# Autodesk Inventor assembly: BG301_trajan20_21
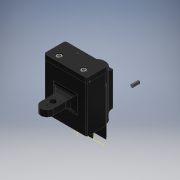
[picture p0: Inventor's stored thumbnail of the model, 180x180]
Saved by Autodesk Inventor 2022.2 (Build 262287000, 287)
## iProperties
Company: HTBLA Kaindorf
RuleStatus: InUse
Created: 2022-08-19
Part Number: BG301_trajan20_21
Project: Zeichenmaschine_v2
Material: Generisch
Description: Stifthalter
Document SubType Name: Assembly
Designer: trajan20
AfterDocNew0: iProperties-Editor_aufrufen
Author: jan
Keywords: 2021
## Documents named in this file (7)
- C:\Users\jan\Documents\DrawMachine\DrawMachineConstruction\Projekt\Zeichenmaschine_v2\BG301_trajan20_21_Zeichenmaschine_v2_Stifthalter.iam
- C:\Users\jan\Documents\DrawMachine\DrawMachineConstruction\Projekt\Zeichenmaschine_v2\BT501_trajan20_21_Zeichenmaschine_v2_Stifthalter außen.ipt
- C:\Users\jan\Documents\DrawMachine\DrawMachineConstruction\Projekt\Zeichenmaschine_v2\BT502_trajan20_21_Zeichenmaschine_v2_Stifthalter innen.ipt
- C:\Users\jan\Documents\DrawMachine\DrawMachineConstruction\Projekt\Zeichenmaschine_v2\BT504_trajan20_21_Zeichenmaschine_v2_Stifthalter_feder.ipt
- C:\Users\jan\Documents\DrawMachine\DrawMachineConstruction\Projekt\Zeichenmaschine_v2\BT503_trajan20_21_Zeichenmaschine_v2_Stifthalter_platte.ipt
- C:\Users\jan\Documents\DrawMachine\DrawMachineConstruction\Projekt\Zeichenmaschine_v2\Normteile\de-DE\ISO 4762(2)\ISO 4762 - M5 x 12ISO.ipt
- C:\Users\jan\Documents\DrawMachine\DrawMachineConstruction\Projekt\Zeichenmaschine_v2\Normteile\de-DE\ISO 4029\ISO 4029 - M5 x 12 - ISO.ipt
## Components (8 placed, 6 different names)
1. BT501_trajan20_21_Zeichenmaschine_v2_Stifthalter außen:1 — Passend:1, Passend:2, Passend:7, Passend:8, Passend:9
2. BT502_trajan20_21_Zeichenmaschine_v2_Stifthalter innen:1 — Passend:1, Passend:2, Passend:3, Passend:4, Passend:5, Passend:6, Passend:11
3. BT504_trajan20_21_Zeichenmaschine_v2_Stifthalter_feder:1 — Passend:3, Passend:6
4. BT504_trajan20_21_Zeichenmaschine_v2_Stifthalter_feder:2 — Passend:4, Passend:5, Passend:10
5. BT503_trajan20_21_Zeichenmaschine_v2_Stifthalter_platte:1 — Passend:7, Passend:8, Passend:9, Passend:10, Einfügen:1, Einfügen:2
6. ISO 4762 M5 x 12:1 — Einfügen:1
7. ISO 4762 M5 x 12:2 — Einfügen:2
8. ISO 4029 M5 x 12:1 — Passend:11
## Relationships (13: Mate 11, Insert 2)
- Passend:1 [Mate]: BT501_trajan20_21_Zeichenmaschine_v2_Stifthalter außen:1 ↔ BT502_trajan20_21_Zeichenmaschine_v2_Stifthalter innen:1
- Passend:2 [Mate]: BT501_trajan20_21_Zeichenmaschine_v2_Stifthalter außen:1 ↔ BT502_trajan20_21_Zeichenmaschine_v2_Stifthalter innen:1
- Passend:3 [Mate]: BT502_trajan20_21_Zeichenmaschine_v2_Stifthalter innen:1 ↔ BT504_trajan20_21_Zeichenmaschine_v2_Stifthalter_feder:1
- Passend:4 [Mate]: BT502_trajan20_21_Zeichenmaschine_v2_Stifthalter innen:1 ↔ BT504_trajan20_21_Zeichenmaschine_v2_Stifthalter_feder:2
- Passend:5 [Mate]: BT502_trajan20_21_Zeichenmaschine_v2_Stifthalter innen:1 ↔ BT504_trajan20_21_Zeichenmaschine_v2_Stifthalter_feder:2
- Passend:6 [Mate]: BT502_trajan20_21_Zeichenmaschine_v2_Stifthalter innen:1 ↔ BT504_trajan20_21_Zeichenmaschine_v2_Stifthalter_feder:1
- Passend:7 [Mate]: BT501_trajan20_21_Zeichenmaschine_v2_Stifthalter außen:1 ↔ BT503_trajan20_21_Zeichenmaschine_v2_Stifthalter_platte:1
- Passend:8 [Mate]: BT501_trajan20_21_Zeichenmaschine_v2_Stifthalter außen:1 ↔ BT503_trajan20_21_Zeichenmaschine_v2_Stifthalter_platte:1
- Passend:9 [Mate]: BT501_trajan20_21_Zeichenmaschine_v2_Stifthalter außen:1 ↔ BT503_trajan20_21_Zeichenmaschine_v2_Stifthalter_platte:1
- Passend:10 [Mate]: BT504_trajan20_21_Zeichenmaschine_v2_Stifthalter_feder:2 ↔ BT503_trajan20_21_Zeichenmaschine_v2_Stifthalter_platte:1
- Einfügen:1 [Insert]: BT503_trajan20_21_Zeichenmaschine_v2_Stifthalter_platte:1 ↔ ISO 4762 M5 x 12:1
- Einfügen:2 [Insert]: BT503_trajan20_21_Zeichenmaschine_v2_Stifthalter_platte:1 ↔ ISO 4762 M5 x 12:2
- Passend:11 [Mate]: BT502_trajan20_21_Zeichenmaschine_v2_Stifthalter innen:1 ↔ ISO 4029 M5 x 12:1
